# Autodesk Inventor assembly: TW-Robot
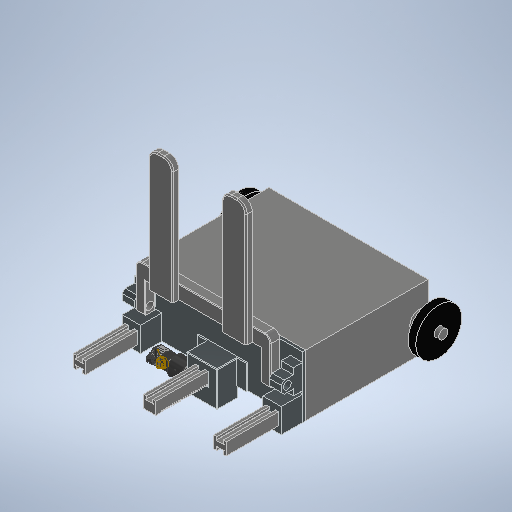
[picture p0: Inventor's stored thumbnail of the model, 512x512]
Saved by Autodesk Inventor 2025.2 (Build 292293000, 293)
## iProperties
Created: 2025-01-03
Part Number: TW-Robot
Document SubType Name: Assembly
Designer: Sergio Quintero
Author: Sergio Quintero
## Documents named in this file (7)
- C:\Users\Sergio Quintero\OneDrive - Universidad Nacional de Colombia\Keio University\Thesis\CAD\TW-Robot.iam
- C:\Users\Sergio Quintero\OneDrive - Universidad Nacional de Colombia\Keio University\Thesis\CAD\Body.ipt
- C:\Users\Sergio Quintero\OneDrive - Universidad Nacional de Colombia\Keio University\Thesis\CAD\Wheel.ipt
- C:\Users\Sergio Quintero\Downloads\CAD\ac-servo-motor-with-planetary-gearbox-hk-kr053g7_05-2.snapshot.2\HG-KR053G7_05\HG-KR053G7_05\HG-KR053G7_05.ipt
- C:\Users\Sergio Quintero\OneDrive - Universidad Nacional de Colombia\Keio University\Thesis\CAD\Lift.ipt
- C:\Users\Sergio Quintero\OneDrive - Universidad Nacional de Colombia\Keio University\Thesis\CAD\Motor_case.ipt
- C:\Users\Sergio Quintero\OneDrive - Universidad Nacional de Colombia\Keio University\Thesis\CAD\Fork.ipt
## Components (7 placed, 6 different names)
1. Body:1 — Rotational:1, Rotational:2, Slider:3
2. Wheel:1 — Rotational:1
3. Wheel:2 — Rotational:2
4. HG-KR053G7_05:1 — Rigid:2
5. Lift:1 — Mate:1, Rigid:4
6. Motor_case:1 — Slider:3, Rigid:2, Mate:1
7. Fork:1 — Rigid:4
## Relationships (6: RevoluteJoint 2, WeldJoint 2, TranslationJoint 1, Mate 1)
- Rotational:1 [RevoluteJoint]: Body:1 ↔ Wheel:1
- Rotational:2 [RevoluteJoint]: Body:1 ↔ Wheel:2
- Slider:3 [TranslationJoint] (5 mm): Body:1 ↔ Motor_case:1
- Rigid:2 [WeldJoint]: HG-KR053G7_05:1 ↔ Motor_case:1
- Mate:1: Lift:1 ↔ Motor_case:1
- Rigid:4 [WeldJoint]: Lift:1 ↔ Fork:1
